# Autodesk Inventor assembly: conveyer_with_sides
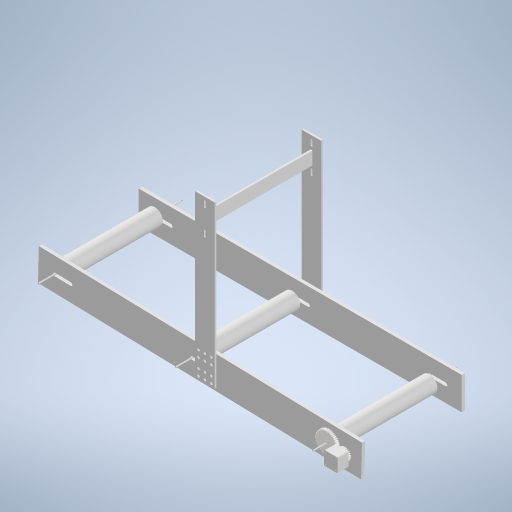
[picture p0: Inventor's stored thumbnail of the model, 512x512]
Saved by Autodesk Inventor 2023 (Build 270158000, 158)
## iProperties
Created: 2022-06-30
Part Number: conveyer_with_sides
Document SubType Name: Assembly
Designer: Zayed
Author: Zayed
## Documents named in this file (9)
- C:\Users\Zayed\Documents\Inventor\Assembly1\conveyer_with_sides.iam
- C:\Users\Zayed\Documents\Inventor\Assembly1\Sides.ipt
- C:\Users\Zayed\Documents\Inventor\Assembly1\Welle.ipt
- C:\Users\Zayed\Documents\Inventor\Assembly1\roller.ipt
- C:\Users\Zayed\Documents\Inventor\Assembly1\Spur Gear24.ipt
- C:\Users\Zayed\Documents\Inventor\Assembly1\Spur Gear14.ipt
- C:\Users\Zayed\Documents\Inventor\Assembly1\motor.ipt
- C:\Users\Zayed\Documents\Inventor\Assembly1\holder_sides.ipt
- C:\Users\Zayed\Documents\Inventor\Assembly1\pi_holder.ipt
## Components (14 placed, 8 different names)
1. Sides:1 — Rotational:1, Rotational:2, Rotational:3, Rotational:4, Rotational:5, Rotational:6, Rotational:7, Mate:3
2. Welle:1 — Rotational:4
3. Welle:2 — Rotational:1
4. Welle:3 — Rotational:2, Mate:4
5. roller:1 — Rotational:3, Mate:1, Mate:2
6. roller:2 — Rotational:5
7. roller:3 — Rotational:6
8. Sides:2 — Mate:1, Mate:2, Flush:2, Mate:10, Mate:11
9. Spur Gear2:1 — Rotational:7
10. Spur Gear1:1 — Mate:3, Mate:4, Mate:5, Mate:6
11. motor:1 — Mate:5, Mate:6
12. holder_sides:2 — Flush:2, Mate:10, Mate:11, Mate:12, Mate:13, Mate:14
13. pi_holder:1 — Mate:12, Mate:13, Mate:14, Mate:15, Mate:16, Mate:17
14. holder_sides:3 — Mate:15, Mate:16, Mate:17
## Relationships (22: Mate 14, RevoluteJoint 7, Flush 1)
- Rotational:1 [RevoluteJoint] (50 mm): Sides:1 ↔ Welle:2
- Rotational:2 [RevoluteJoint] (50 mm): Sides:1 ↔ Welle:3
- Rotational:3 [RevoluteJoint]: Sides:1 ↔ roller:1
- Rotational:4 [RevoluteJoint] (-50 mm): Sides:1 ↔ Welle:1
- Rotational:5 [RevoluteJoint]: Sides:1 ↔ roller:2
- Rotational:6 [RevoluteJoint]: Sides:1 ↔ roller:3
- Mate:1: roller:1 ↔ Sides:2
- Mate:2: roller:1 ↔ Sides:2
- Rotational:7 [RevoluteJoint]: Sides:1 ↔ Spur Gear2:1
- Mate:3: Sides:1 ↔ Spur Gear1:1
- Mate:4 (50 mm): Welle:3 ↔ Spur Gear1:1
- Mate:5: Spur Gear1:1 ↔ motor:1
- Mate:6: Spur Gear1:1 ↔ motor:1
- Flush:2: Sides:2 ↔ holder_sides:2
- Mate:10: Sides:2 ↔ holder_sides:2
- Mate:11 (-29.87 mm): Sides:2 ↔ holder_sides:2
- Mate:12: holder_sides:2 ↔ pi_holder:1
- Mate:13: holder_sides:2 ↔ pi_holder:1
- Mate:14: holder_sides:2 ↔ pi_holder:1
- Mate:15: pi_holder:1 ↔ holder_sides:3
- Mate:16: pi_holder:1 ↔ holder_sides:3
- Mate:17: pi_holder:1 ↔ holder_sides:3
